# Autodesk Inventor assembly: MotorRight
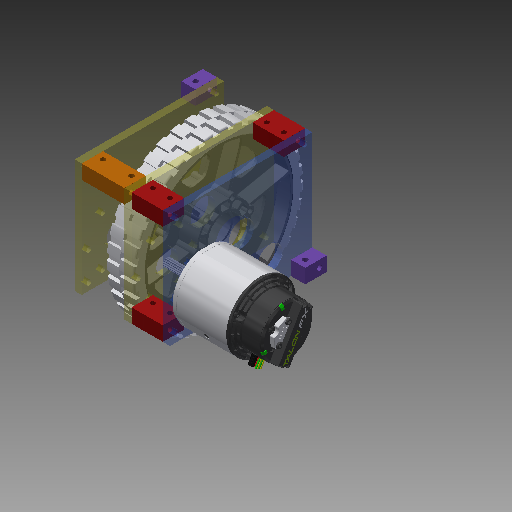
[picture p0: Inventor's stored thumbnail of the model, 512x512]
Saved by Autodesk Inventor 2019 (Build 230136000, 136)
## iProperties
Created: 2020-03-02
Part Number: MotorRight
Document SubType Name: Assembly
Designer: james
Author: james
## Documents named in this file (8)
- F:\JimsRobot\FIRSTRobots\Design\TornadoPlatypus\MotorRight.iam
- F:\JimsRobot\FIRSTRobots\Design\TornadoPlatypus\InsideMotorPlate.ipt
- F:\JimsRobot\FIRSTRobots\Design\Library\CTR\Falcon\217-6515 20191025.iam
- F:\JimsRobot\FIRSTRobots\Design\TornadoPlatypus\MotorSpacerBlock.ipt
- F:\JimsRobot\FIRSTRobots\Design\Library\AndyMark\6 HiGrip Asm Rev II.iam
- F:\JimsRobot\FIRSTRobots\Design\TornadoPlatypus\MotorSpacerBlock2.ipt
- F:\JimsRobot\FIRSTRobots\Design\TornadoPlatypus\MotorSpacerBlock3.ipt
- F:\JimsRobot\FIRSTRobots\Design\TornadoPlatypus\OutsideMotorPlate.ipt
## Components (12 placed, 7 different names)
1. InsideMotorPlate:1 — Mate:1, Mate:2, Mate:3, Mate:4, Mate:6, Mate:7, Mate:8, Flush:1, Mate:9, Flush:2, Mate:11, Flush:4
2. 217-6515 20191025:1 [sub-assembly] — Mate:1, Mate:2, Mate:3
3. MotorSpacerBlock:1 — Mate:7, Mate:9, Flush:2, Mate:24, Mate:25
4. MotorSpacerBlock:2 — Mate:4, Mate:11, Flush:4
5. MotorSpacerBlock:3 — Mate:6, Mate:8, Flush:1, Mate:14
6. OutsideMotorPlate:2 — Mate:14, Mate:15, Mate:16, Mate:17, Mate:18, Flush:5, Mate:21, Mate:24, Mate:25
7. 6 HiGrip Asm Rev II:1 [sub-assembly] — Mate:15, Mate:16
8. MotorSpacerBlock2:1 — Mate:17, Mate:18, Flush:5, Mate:19, Mate:20
9. OutsideMotorPlate:1 — Mate:19, Mate:20, Mate:21, Mate:22, Mate:23, Flush:6, Mate:26, Mate:29, Flush:8
10. MotorSpacerBlock3:1
11. MotorSpacerBlock3:2 — Mate:22, Mate:23, Flush:6
12. MotorSpacerBlock3:4 — Mate:26, Mate:29, Flush:8
## Relationships (29: Mate 23, Flush 6)
- Mate:1: InsideMotorPlate:1 ↔ 217-6515 20191025:1
- Mate:2: InsideMotorPlate:1 ↔ 217-6515 20191025:1
- Mate:3: InsideMotorPlate:1 ↔ 217-6515 20191025:1
- Mate:4: InsideMotorPlate:1 ↔ MotorSpacerBlock:2
- Mate:6: InsideMotorPlate:1 ↔ MotorSpacerBlock:3
- Mate:7: InsideMotorPlate:1 ↔ MotorSpacerBlock:1
- Mate:8: InsideMotorPlate:1 ↔ MotorSpacerBlock:3
- Flush:1: InsideMotorPlate:1 ↔ MotorSpacerBlock:3
- Mate:9: InsideMotorPlate:1 ↔ MotorSpacerBlock:1
- Flush:2: InsideMotorPlate:1 ↔ MotorSpacerBlock:1
- Mate:11: InsideMotorPlate:1 ↔ MotorSpacerBlock:2
- Flush:4: InsideMotorPlate:1 ↔ MotorSpacerBlock:2
- Mate:14: MotorSpacerBlock:3 ↔ OutsideMotorPlate:2
- Mate:15: OutsideMotorPlate:2 ↔ 6 HiGrip Asm Rev II:1
- Mate:16: OutsideMotorPlate:2 ↔ 6 HiGrip Asm Rev II:1
- Mate:17: OutsideMotorPlate:2 ↔ MotorSpacerBlock2:1
- Mate:18: OutsideMotorPlate:2 ↔ MotorSpacerBlock2:1
- Flush:5: OutsideMotorPlate:2 ↔ MotorSpacerBlock2:1
- Mate:19: MotorSpacerBlock2:1 ↔ OutsideMotorPlate:1
- Mate:20: MotorSpacerBlock2:1 ↔ OutsideMotorPlate:1
- Mate:21: OutsideMotorPlate:2 ↔ OutsideMotorPlate:1
- Mate:22: OutsideMotorPlate:1 ↔ MotorSpacerBlock3:2
- Mate:23: OutsideMotorPlate:1 ↔ MotorSpacerBlock3:2
- Flush:6: OutsideMotorPlate:1 ↔ MotorSpacerBlock3:2
- Mate:24: MotorSpacerBlock:1 ↔ OutsideMotorPlate:2
- Mate:25: MotorSpacerBlock:1 ↔ OutsideMotorPlate:2
- Mate:26: OutsideMotorPlate:1 ↔ MotorSpacerBlock3:4
- Mate:29: OutsideMotorPlate:1 ↔ MotorSpacerBlock3:4
- Flush:8: OutsideMotorPlate:1 ↔ MotorSpacerBlock3:4
